# Autodesk Inventor assembly: GATITOLOCO
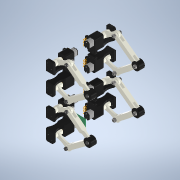
[picture p0: Inventor's stored thumbnail of the model, 180x180]
Saved by Autodesk Inventor 2022 (Build 260153000, 153)
## iProperties
Created: 2021-12-08
Part Number: GATITOLOCO
Document SubType Name: Assembly
Designer: JK
Author: JK
## Documents named in this file (3)
- C:\Users\JK\Documents\Inventor\N20 Leg Actuator\N20-Leg-Actuator\CADfiles\GATITOLOCO\GATITOLOCO.iam
- C:\Users\JK\Documents\Inventor\N20 Leg Actuator\N20-Leg-Actuator\CADfiles\N20 Leg\LegAssembly.iam
- C:\Users\JK\Documents\Inventor\N20 Leg Actuator\N20-Leg-Actuator\CADfiles\GATITOLOCO\Electronics\Teensy4.iam
## Components (5 placed, 2 different names)
1. LegAssembly:1 [sub-assembly] — Nivelación:1, Nivelación:2, Ángulo:1, Nivelación:3, Nivelación:7
2. LegAssembly:2 [sub-assembly] — Ángulo:1, Nivelación:3, Nivelación:5, Nivelación:6, Nivelación:7
3. LegAssembly:3 [sub-assembly] — Nivelación:1, Nivelación:2, Nivelación:4
4. LegAssembly:4 [sub-assembly] — Nivelación:4, Nivelación:5, Nivelación:6
5. Teensy4:1 [sub-assembly]
## Relationships (8: Flush 7, Angle 1)
- Nivelación:1 [Flush]: LegAssembly:1 ↔ LegAssembly:3
- Nivelación:2 [Flush]: LegAssembly:1 ↔ LegAssembly:3
- Ángulo:1 [Angle] (180 deg): LegAssembly:1 ↔ LegAssembly:2
- Nivelación:3 [Flush]: LegAssembly:1 ↔ LegAssembly:2
- Nivelación:4 [Flush]: LegAssembly:3 ↔ LegAssembly:4
- Nivelación:5 [Flush]: LegAssembly:2 ↔ LegAssembly:4
- Nivelación:6 [Flush]: LegAssembly:2 ↔ LegAssembly:4
- Nivelación:7 [Flush]: LegAssembly:1 ↔ LegAssembly:2
